# Autodesk Inventor assembly: Сборка1
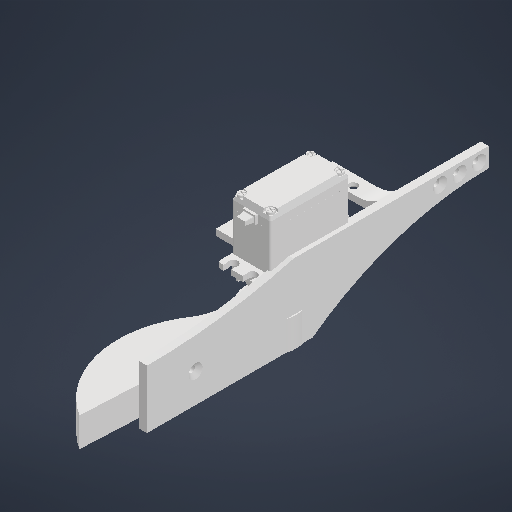
[picture p0: Inventor's stored thumbnail of the model, 512x512]
Saved by Autodesk Inventor 2025 (Build 290162000, 162)
## iProperties
Created: 2024-11-13
Part Number: Сборка1
Document SubType Name: Assembly
Designer: Phantom
Author: Phantom
## Documents named in this file (4)
- C:\Users\Phantom\Desktop\Phantom16950\Сборка1.iam
- C:\Users\Phantom\Desktop\Phantom16950\2000-0025-0002\2000-0025-0002.ipt
- C:\Users\Phantom\Desktop\Phantom16950\клешня сос.ipt
- C:\Users\Phantom\Desktop\Phantom16950\хрень.ipt
## Components (3 placed, 3 different names)
1. 2000-0025-0002:1 — Совмещение:1, Совмещение:2, Совмещение:3
2. клешня сос:1 — Совмещение:1
3. хрень:1 — Совмещение:2, Совмещение:3
## Relationships (3: Mate 3)
- Совмещение:1 [Mate]: 2000-0025-0002:1 ↔ клешня сос:1
- Совмещение:2 [Mate]: 2000-0025-0002:1 ↔ хрень:1
- Совмещение:3 [Mate] (4 mm): 2000-0025-0002:1 ↔ хрень:1
